# Autodesk Inventor assembly: 16mm_Tube_Connector_MIR
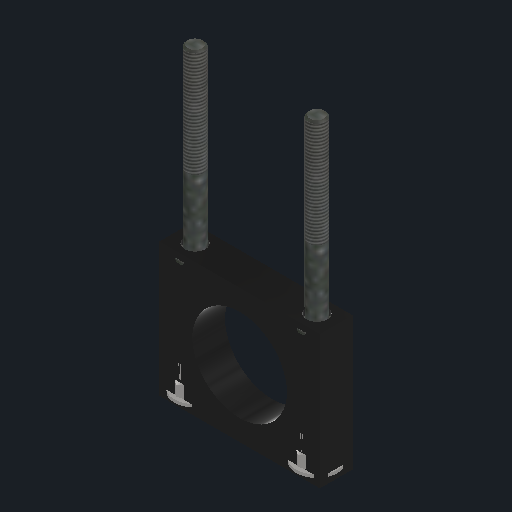
[picture p0: Inventor's stored thumbnail of the model, 512x512]
Saved by Autodesk Inventor 2024.1 (Build 281209000, 209)
## iProperties
Created: 2023-12-04
Part Number: 16mm_Tube_Connector_MIR
Document SubType Name: Assembly
Designer: dzw04
Author: dzw04
## Documents named in this file (5)
- C:\Users\dzw04\Saxion\Mechatronica Lectoraat LMECH LED - Database ARG\Component_Database\SARAX\01. CAD\01. 3D_Drawing\02. Sub_Assemblies\Landing_Gear\02. Sub_Assemblies\16mm_Tube_Connector_MIR.iam
- C:\Users\dzw04\Saxion\Mechatronica Lectoraat LMECH LED - Database ARG\Component_Database\SARAX\01. CAD\01. 3D_Drawing\02. Sub_Assemblies\Landing_Gear\01. Parts\16mm_Tube_Connecotor_Holybro_MIR.ipt
- C:\Users\dzw04\OneDrive - Saxion\Documenten\Inventor\Content Center Files\R2024\en-US\ISO 7380-1\ISO 7380-1 - M3 x 30.ipt
- C:\Users\dzw04\OneDrive - Saxion\Documenten\Inventor\Content Center Files\R2024\en-US\ISO 7089\ISO 7089 - 3 - 140 HV(1).ipt
- C:\Users\dzw04\OneDrive - Saxion\Documenten\Inventor\Content Center Files\R2024\en-US\NF E 25-409\NF E 25-409 - M3.ipt
## Components (8 placed, 4 different names)
1. 16mm_Tube_Connecotor_Holybro_MIR:1 — Flush:2, Flush:1, Mate:1, Mate:4
2. 16mm_Tube_Connecotor_Holybro_MIR:2 — Flush:2, Flush:1, Mate:1, Mate:3, Mate:2
3. ISO 7380-1 M3 x 30:1 — Mate:3, Mate:2, Mate:5, Mate:7
4. ISO 7089 3:1 — Mate:5, Mate:4, Mate:6
5. NF E 25-409 M3:1 — Mate:7, Mate:6
6. ISO 7380-1 M3 x 30:2
7. ISO 7089 3:2
8. NF E 25-409 M3:2
## Component patterns: (2 elements, first: ISO 7380-1 M3 x 30:1 + ISO 7089 3:1 + NF E 25-409 M3:1)
## Relationships (9: Mate 7, Flush 2)
- Flush:2: 16mm_Tube_Connecotor_Holybro_MIR:1 ↔ 16mm_Tube_Connecotor_Holybro_MIR:2
- Flush:1: 16mm_Tube_Connecotor_Holybro_MIR:1 ↔ 16mm_Tube_Connecotor_Holybro_MIR:2
- Mate:1: 16mm_Tube_Connecotor_Holybro_MIR:1 ↔ 16mm_Tube_Connecotor_Holybro_MIR:2
- Mate:3: 16mm_Tube_Connecotor_Holybro_MIR:2 ↔ ISO 7380-1 M3 x 30:1
- Mate:2 (1 mm): 16mm_Tube_Connecotor_Holybro_MIR:2 ↔ ISO 7380-1 M3 x 30:1
- Mate:5: ISO 7380-1 M3 x 30:1 ↔ ISO 7089 3:1
- Mate:4 (1 mm): 16mm_Tube_Connecotor_Holybro_MIR:1 ↔ ISO 7089 3:1
- Mate:7: ISO 7380-1 M3 x 30:1 ↔ NF E 25-409 M3:1
- Mate:6: ISO 7089 3:1 ↔ NF E 25-409 M3:1
